# Autodesk Inventor assembly: Needle Roller Assembly
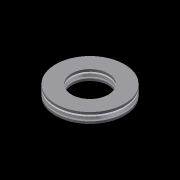
[picture p0: Inventor's stored thumbnail of the model, 180x180]
Saved by Autodesk Inventor 2014 SP1 (Build 180222100, 222)
## iProperties
Created: 2014-05-04
Part Number: Needle Roller Assembly
Document SubType Name: Assembly
Designer: Rauhul Varma
Author: Rauhul Varma
## Documents named in this file (3)
- C:\Users\Rauhul Varma\Desktop\GRT 2013-2014 Designs\Low CoG Swerve\Needle Roller Assembly.iam
- C:\Users\Rauhul Varma\Desktop\GRT 2013-2014 Designs\Low CoG Swerve\.5000 ID Needle Roller Washer.ipt
- C:\Users\Rauhul Varma\Desktop\GRT 2013-2014 Designs\Low CoG Swerve\.5000 ID Needle Roller Thrust Bearing.ipt
## Components (3 placed, 2 different names)
1. .5000 ID Needle Roller Washer:1 — Tangent:1, Mate:1, Mate:2
2. .5000 ID Needle Roller Thrust Bearing:1 — Tangent:1, Mate:1, Mate:2, Mate:3, Mate:4
3. .5000 ID Needle Roller Washer:2 — Mate:3, Mate:4
## Relationships (5: Mate 4, Tangent 1)
- Tangent:1: .5000 ID Needle Roller Washer:1 ↔ .5000 ID Needle Roller Thrust Bearing:1
- Mate:1: .5000 ID Needle Roller Washer:1 ↔ .5000 ID Needle Roller Thrust Bearing:1
- Mate:2 (0.4961 mm): .5000 ID Needle Roller Washer:1 ↔ .5000 ID Needle Roller Thrust Bearing:1
- Mate:3 (0.4961 mm): .5000 ID Needle Roller Thrust Bearing:1 ↔ .5000 ID Needle Roller Washer:2
- Mate:4: .5000 ID Needle Roller Thrust Bearing:1 ↔ .5000 ID Needle Roller Washer:2
